# Autodesk Inventor assembly: Camera Gimble
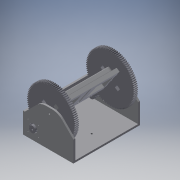
[picture p0: Inventor's stored thumbnail of the model, 180x180]
Saved by Autodesk Inventor 2016 (Build 200138000, 138)
## iProperties
Created: 2016-11-04
Part Number: Camera Gimble
Document SubType Name: Assembly
Designer: william
Author: william
## Documents named in this file (8)
- C:\Users\William\Dropbox\Projects\0052 - Camera Gimble\Camera Gimble.iam
- C:\Users\William\Dropbox\Projects\0052 - Camera Gimble\Base Plate.ipt
- C:\Users\William\Dropbox\Projects\0052 - Camera Gimble\Side Plate.ipt
- C:\Users\William\Dropbox\Projects\0052 - Camera Gimble\Back Plate.ipt
- C:\Users\William\Dropbox\Projects\0052 - Camera Gimble\Samsung S5.ipt
- C:\Users\William\Dropbox\Projects\0052 - Camera Gimble\Camera Gimble\Design Accelerator\Spur Gears1.iam
- C:\Users\William\Dropbox\Projects\0052 - Camera Gimble\center mount.ipt
- C:\Users\William\Dropbox\Projects\0052 - Camera Gimble\17HM19-2004S\17HM19-2004S.iam
## Components (9 placed, 7 different names)
1. Base Plate:1 — Rigid:7
2. Side Plate:2 — Rotational:1, Rotational:2, Rigid:7, Rigid:8
3. Back Plate:1 — Rigid:8, Rotational:4
4. Samsung S5:1
5. Spur Gears:1 [sub-assembly] — Rigid:5, Rotational:1
6. center mount:1 — Rigid:5, Rotational:3
7. 17HM19-2004S:1 [sub-assembly] — Rotational:2
8. Spur Gears:2 [sub-assembly] — Rotational:3
9. Side Plate:3 — Rotational:4
## Relationships (7: RevoluteJoint 4, WeldJoint 3)
- Rigid:5 [WeldJoint]: Spur Gears:1 ↔ center mount:1
- Rotational:1 [RevoluteJoint]: Side Plate:2 ↔ Spur Gears:1
- Rotational:2 [RevoluteJoint]: Side Plate:2 ↔ 17HM19-2004S:1
- Rigid:7 [WeldJoint]: Base Plate:1 ↔ Side Plate:2
- Rigid:8 [WeldJoint]: Side Plate:2 ↔ Back Plate:1
- Rotational:3 [RevoluteJoint]: center mount:1 ↔ Spur Gears:2
- Rotational:4 [RevoluteJoint]: Back Plate:1 ↔ Side Plate:3
